# Autodesk Inventor assembly: Intake motor on xrail
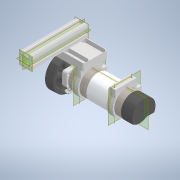
[picture p0: Inventor's stored thumbnail of the model, 180x180]
Saved by Autodesk Inventor 2020 (Build 240168000, 168)
## iProperties
Created: 2020-01-13
Part Number: Intake motor on xrail
Document SubType Name: Assembly
Designer: ball
Author: ball
## Documents named in this file (5)
- D:\FTC8863\2019 Robot\Collection\Intake motor on xrail.iam
- D:\FTC8863\2019 Robot\Collection\neverest 40 + mounts.iam
- D:\FTC8863\2019 Robot\Collection\compliant wheel 2 in + 6mm shaft adapterr.iam
- D:\FTC8863\Actobotics\565 parts\xrail_3.5in.ipt
- D:\FTC8863\2019 Robot\Collection\intake motor mount to xrail.ipt
## Components (4 placed, 4 different names)
1. neverest 40 + mounts:1 [sub-assembly] — Flush:3
2. compliant wheel 2 in + 6mm shaft adapterr:1 [sub-assembly]
3. xrail_3.5in:1 — Flush:4
4. intake motor mount to xrail:1 — Flush:3, Flush:4
## Relationships (7: Mate 4, Flush 3)
- [Mate]: neverest 40 + mounts:1 ↔ compliant wheel 2 in + 6mm shaft adapterr:1
- [Mate]: neverest 40 + mounts:1 ↔ compliant wheel 2 in + 6mm shaft adapterr:1
- [Mate]: xrail_3.5in:1 ↔ intake motor mount to xrail:1
- [Flush]: xrail_3.5in:1 ↔ intake motor mount to xrail:1
- [Mate]: neverest 40 + mounts:1 ↔ intake motor mount to xrail:1
- Flush:3 (-5.08 mm): neverest 40 + mounts:1 ↔ intake motor mount to xrail:1
- Flush:4: xrail_3.5in:1 ↔ intake motor mount to xrail:1
